# Autodesk Inventor assembly: RoArm_ensamble
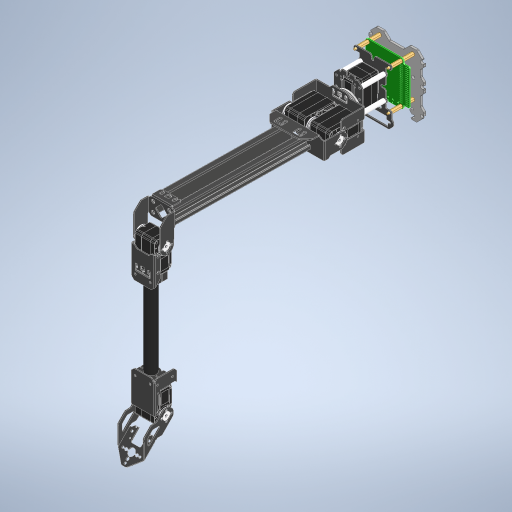
[picture p0: Inventor's stored thumbnail of the model, 512x512]
Saved by Autodesk Inventor 2024.4 (Build 284460000, 460)
## iProperties
Created: 2026-06-03
Part Number: RoArm_ensamble
Document SubType Name: Assembly
Designer: epm01
Author: epm01
## Documents named in this file (6)
- D:\Archivos\2026-2\RoArm\inventor\RoArm_ensamble.iam
- D:\Archivos\2026-2\RoArm\inventor\RoArm_base_link.iam
- D:\Archivos\2026-2\RoArm\inventor\RoArm_cintura.iam
- D:\Archivos\2026-2\RoArm\inventor\RoArm_antebrazo.iam
- D:\Archivos\2026-2\RoArm\inventor\RoArm_brazo.iam
- D:\Archivos\2026-2\RoArm\inventor\AL_grippe.ipt
## Components (5 placed, 5 different names)
1. RoArm_base_link:1 [sub-assembly] — Rotational:1
2. RoArm_cintura:1 [sub-assembly] — Rotational:1, Rotational:2
3. RoArm_antebrazo:1 [sub-assembly] — Rotational:2, Rotational:3
4. RoArm_brazo:1 [sub-assembly] — Rotational:3, Rotational:4
5. AL_grippe:1 — Rotational:4
## Relationships (4: RevoluteJoint 4)
- Rotational:1 [RevoluteJoint]: RoArm_base_link:1 ↔ RoArm_cintura:1
- Rotational:2 [RevoluteJoint]: RoArm_cintura:1 ↔ RoArm_antebrazo:1
- Rotational:3 [RevoluteJoint]: RoArm_antebrazo:1 ↔ RoArm_brazo:1
- Rotational:4 [RevoluteJoint]: RoArm_brazo:1 ↔ AL_grippe:1
